# Autodesk Inventor assembly: gear support + attachment
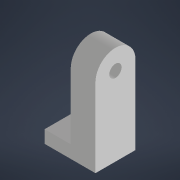
[picture p0: Inventor's stored thumbnail of the model, 180x180]
Saved by Autodesk Inventor 2022 (Build 260153000, 153)
## iProperties
Created: 2022-01-26
Part Number: gear support + attachment
Document SubType Name: Assembly
Designer: gordo
Author: gordo
## Documents named in this file (3)
- C:\Users\gordo\OneDrive\Documents\Inventor Projects\project 3\gear support + attachment.iam
- C:\Users\gordo\OneDrive\Documents\Inventor Projects\project 3\gear support attachment.ipt
- C:\Users\gordo\OneDrive\Documents\Inventor Projects\project 3\gear support.ipt
## Components (2 placed, 2 different names)
1. gear support attachment:1 — Mate:1, Flush:1, Flush:2
2. gear support:1 — Mate:1, Flush:1, Flush:2
## Relationships (3: Flush 2, Mate 1)
- Mate:1: gear support attachment:1 ↔ gear support:1
- Flush:1: gear support attachment:1 ↔ gear support:1
- Flush:2: gear support attachment:1 ↔ gear support:1
